# Autodesk Inventor assembly: 프레임조립
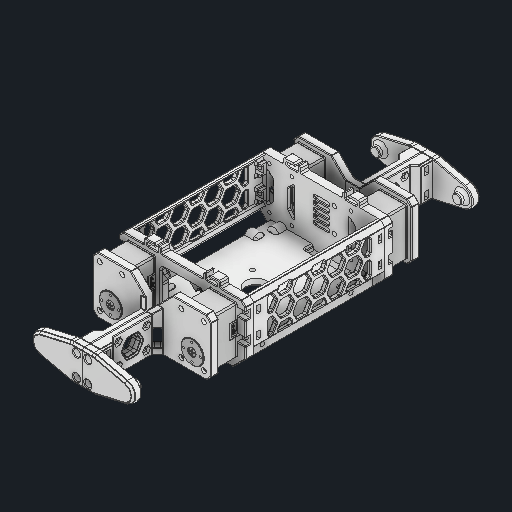
[picture p0: Inventor's stored thumbnail of the model, 512x512]
Saved by Autodesk Inventor 2027.1 (Build 311270010, 270A)
## iProperties
Created: 2026-08-10
Part Number: 프레임조립
Document SubType Name: Assembly
Designer: moieboy9999
Mass: 220.643 g
Surface Area: 1298.42 cm^2
Volume: 188.594 cm^3
Density: 1.16994 g/cm^3
Author: moieboy9999
## Documents named in this file (9)
- D:\micro_dog_cad\몸\프레임\프레임조립.iam
- D:\micro_dog_cad\몸\프레임\아래프레임.ipt
- D:\micro_dog_cad\몸\프레임\사이드프레임.ipt
- D:\micro_dog_cad\몸\프레임\뒷프레임.ipt
- D:\micro_dog_cad\몸\프레임\앞프레임.ipt
- D:\micro_dog_cad\부품\XL,XC-330.ipt
- D:\micro_dog_cad\몸\프레임\롤축지지대.ipt
- D:\micro_dog_cad\몸\프레임\롤축지지대_MIR.ipt
- D:\micro_dog_cad\몸\프레임\롤축지지대베어링.ipt
## Components (17 placed, 8 different names)
1. 뒷프레임:1 — 메이트:8, 메이트:11, 메이트:12, 메이트:13, 메이트:15, 플러쉬:1, 메이트:41
2. 앞프레임:1 — 메이트:7, 메이트:9, 메이트:10, 메이트:14, 메이트:16, 메이트:38, 메이트:39, 메이트:40, 메이트:42
3. 아래프레임:1 — 메이트:7, 메이트:8, 메이트:17, 메이트:18, 메이트:40
4. XL,XC-330:1 — 메이트:11, 메이트:15, 메이트:25, 메이트:26
5. XL,XC-330:2 — 메이트:12, 메이트:13, 메이트:22, 메이트:27
6. XL,XC-330:3 — 메이트:9, 메이트:14, 메이트:28, 메이트:29
7. XL,XC-330:4 — 메이트:10, 메이트:16, 메이트:23, 메이트:24
8. 롤축지지대:1 — 메이트:28, 메이트:29, 메이트:34, 메이트:36
9. 롤축지지대:2 — 메이트:22, 메이트:27, 메이트:30, 메이트:31
10. 롤축지지대_MIR:1 — 메이트:23, 메이트:24, 메이트:35, 메이트:37
11. 롤축지지대_MIR:2 — 메이트:25, 메이트:26, 메이트:32, 메이트:33
12. 롤축지지대베어링:1 — 메이트:32, 메이트:33
13. 롤축지지대베어링:2 — 메이트:30, 메이트:31
14. 롤축지지대베어링:3 — 메이트:35, 메이트:37
15. 롤축지지대베어링:4 — 메이트:34, 메이트:36
16. 사이드프레임:1 — 메이트:38, 메이트:39
17. 사이드프레임:2 — 메이트:41, 메이트:42
## Relationships (34: Mate 33, Flush 1)
- 메이트:7 [Mate]: 앞프레임:1 ↔ 아래프레임:1
- 메이트:8 [Mate]: 뒷프레임:1 ↔ 아래프레임:1
- 메이트:9 [Mate]: 앞프레임:1 ↔ XL,XC-330:3
- 메이트:10 [Mate]: 앞프레임:1 ↔ XL,XC-330:4
- 메이트:11 [Mate]: 뒷프레임:1 ↔ XL,XC-330:1
- 메이트:12 [Mate]: 뒷프레임:1 ↔ XL,XC-330:2
- 메이트:13 [Mate]: 뒷프레임:1 ↔ XL,XC-330:2
- 메이트:14 [Mate]: 앞프레임:1 ↔ XL,XC-330:3
- 메이트:15 [Mate]: 뒷프레임:1 ↔ XL,XC-330:1
- 메이트:16 [Mate]: 앞프레임:1 ↔ XL,XC-330:4
- 메이트:17 [Mate]: 아래프레임:1
- 메이트:18 [Mate]: 아래프레임:1
- 플러쉬:1 [Flush]: 뒷프레임:1
- 메이트:22 [Mate]: XL,XC-330:2 ↔ 롤축지지대:2
- 메이트:23 [Mate]: XL,XC-330:4 ↔ 롤축지지대_MIR:1
- 메이트:24 [Mate]: XL,XC-330:4 ↔ 롤축지지대_MIR:1
- 메이트:25 [Mate]: XL,XC-330:1 ↔ 롤축지지대_MIR:2
- 메이트:26 [Mate]: XL,XC-330:1 ↔ 롤축지지대_MIR:2
- 메이트:27 [Mate]: XL,XC-330:2 ↔ 롤축지지대:2
- 메이트:28 [Mate]: XL,XC-330:3 ↔ 롤축지지대:1
- 메이트:29 [Mate]: XL,XC-330:3 ↔ 롤축지지대:1
- 메이트:30 [Mate]: 롤축지지대:2 ↔ 롤축지지대베어링:2
- 메이트:31 [Mate]: 롤축지지대:2 ↔ 롤축지지대베어링:2
- 메이트:32 [Mate]: 롤축지지대_MIR:2 ↔ 롤축지지대베어링:1
- 메이트:33 [Mate]: 롤축지지대_MIR:2 ↔ 롤축지지대베어링:1
- 메이트:34 [Mate]: 롤축지지대:1 ↔ 롤축지지대베어링:4
- 메이트:35 [Mate]: 롤축지지대_MIR:1 ↔ 롤축지지대베어링:3
- 메이트:36 [Mate]: 롤축지지대:1 ↔ 롤축지지대베어링:4
- 메이트:37 [Mate]: 롤축지지대_MIR:1 ↔ 롤축지지대베어링:3
- 메이트:38 [Mate]: 앞프레임:1 ↔ 사이드프레임:1
- 메이트:39 [Mate]: 앞프레임:1 ↔ 사이드프레임:1
- 메이트:40 [Mate]: 앞프레임:1 ↔ 아래프레임:1
- 메이트:41 [Mate]: 뒷프레임:1 ↔ 사이드프레임:2
- 메이트:42 [Mate]: 앞프레임:1 ↔ 사이드프레임:2
